# Autodesk Inventor assembly: ZMotorassembly
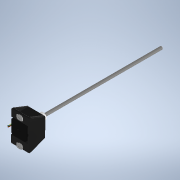
[picture p0: Inventor's stored thumbnail of the model, 180x180]
Saved by Autodesk Inventor 2020.2 (Build 242310000, 310)
## iProperties
Created: 2020-08-25
Part Number: ZMotorassembly
Document SubType Name: Assembly
Designer: JK
Author: JK
## Documents named in this file (8)
- C:\Users\JK\Documents\Inventor\Anet Upgrade\ZMotorassembly.iam
- C:\Users\JK\Documents\Inventor\Anet Upgrade\MOTOR.ipt
- C:\Users\JK\Documents\Inventor\Anet Upgrade\zmotorsupport.ipt
- C:\Users\JK\Documents\Inventor\Anet Upgrade\M3x10.ipt
- C:\Users\JK\Documents\Inventor\Anet Upgrade\ACMEThread.ipt
- C:\Users\JK\Documents\Inventor\Anet Upgrade\T_Slot_Nut_Dropin_3030m5ipt.ipt
- C:\Users\JK\Documents\Inventor\Anet Upgrade\M5x8BoltFlatHead.ipt
- C:\Users\JK\Documents\Inventor\Anet Upgrade\Flexible_Shaft_Coupling_5_to_8mm v7.iam
## Components (12 placed, 7 different names)
1. MOTOR:1 — Angle:1, Mate:8, Mate:9, Mate:16
2. zmotorsupport:1 — Angle:1, Mate:3, Mate:4, Mate:5, Mate:6, Mate:7, Mate:10, Mate:11, Mate:12, Angle:2, Angle:3, Mate:15, Mate:17
3. M3x10:1 — Mate:5, Flush:2, Flush:3, Mate:7
4. M3x10:2 — Mate:4, Flush:3
5. M3x10:3 — Mate:3, Flush:1
6. M3x10:4 — Mate:6, Flush:1, Flush:2
7. Wał:1 — Mate:8, Mate:9
8. M5x8BoltFlatHead:1 — Mate:11, Flush:4, Mate:14
9. M5x8BoltFlatHead:2 — Mate:10, Flush:4, Mate:12, Mate:13
10. T_Slot_Nut_Dropin_3030m5ipt:1 — Mate:14, Angle:3, Flush:5
11. T_Slot_Nut_Dropin_3030m5ipt:2 — Mate:13, Angle:2, Flush:5, Mate:15
12. Flexible_Shaft_Coupling_5_to_8mm v7:1 [sub-assembly] — Mate:16, Mate:17
## Relationships (25: Mate 17, Flush 5, Angle 3)
- [Mate]: MOTOR:1 ↔ zmotorsupport:1
- Angle:1 (90 deg): MOTOR:1 ↔ zmotorsupport:1
- [Mate]: MOTOR:1 ↔ zmotorsupport:1
- Mate:3: zmotorsupport:1 ↔ M3x10:3
- Mate:4: zmotorsupport:1 ↔ M3x10:2
- Mate:5: zmotorsupport:1 ↔ M3x10:1
- Mate:6: zmotorsupport:1 ↔ M3x10:4
- Flush:1: M3x10:3 ↔ M3x10:4
- Flush:2: M3x10:1 ↔ M3x10:4
- Flush:3: M3x10:1 ↔ M3x10:2
- Mate:7: zmotorsupport:1 ↔ M3x10:1
- Mate:8: MOTOR:1 ↔ Wał:1
- Mate:9: MOTOR:1 ↔ Wał:1
- Mate:10: zmotorsupport:1 ↔ M5x8BoltFlatHead:2
- Mate:11: zmotorsupport:1 ↔ M5x8BoltFlatHead:1
- Flush:4: M5x8BoltFlatHead:1 ↔ M5x8BoltFlatHead:2
- Mate:12: zmotorsupport:1 ↔ M5x8BoltFlatHead:2
- Mate:13: M5x8BoltFlatHead:2 ↔ T_Slot_Nut_Dropin_3030m5ipt:2
- Mate:14: M5x8BoltFlatHead:1 ↔ T_Slot_Nut_Dropin_3030m5ipt:1
- Angle:2 (0 deg): zmotorsupport:1 ↔ T_Slot_Nut_Dropin_3030m5ipt:2
- Angle:3 (0 deg): zmotorsupport:1 ↔ T_Slot_Nut_Dropin_3030m5ipt:1
- Flush:5: T_Slot_Nut_Dropin_3030m5ipt:1 ↔ T_Slot_Nut_Dropin_3030m5ipt:2
- Mate:15: zmotorsupport:1 ↔ T_Slot_Nut_Dropin_3030m5ipt:2
- Mate:16: MOTOR:1 ↔ Flexible_Shaft_Coupling_5_to_8mm v7:1
- Mate:17 (-1 mm): zmotorsupport:1 ↔ Flexible_Shaft_Coupling_5_to_8mm v7:1
